# Autodesk Inventor assembly: 6_right_arm_no error
(part 2 of 2)
Size Designation: M3 x 6
Categories: <MemberInstance><Categories><Category DisplayName="Fasteners" InternalName="e4da775c-781d-43d5-af7c-5136215cf5a6" Mnemonic="FSTN"><Category DisplayName="Bolts" InternalName="536e6df0-f778-49ac-b2f2-25c71d2aa0b2" Mnemonic="SCRW"><CategoryParameter DisplayName="Nominal Diameter Designation" InternalName="03caf894-eafd-4c09-a035-916ac084b87b" Mnemonic="nomdiadesig"/><CategoryParameter DisplayName="Nominal Length" InternalName="238ecbaf-3e6c-45dd-aa95-4068c8e0fd02" Mnemonic="nomlen"/><CategoryParameter DisplayName="Thread Designation" InternalName="586d5e89-370a-4089-914f-0110033585c7" Mnemonic="thrdesign"/><CategoryParameter DisplayName="Thread Series Designation" InternalName="87c5849c-b3a5-4c3e-9c9b-2feecef9be86" Mnemonic="thrserdsgn"/><CategoryParameter DisplayName="Nominal Diameter" InternalName="8bbe3f8e-44cf-40a9-a251-3a6edc8168d6" Mnemonic="nomdia"/><CategoryParameter DisplayName="Thread Type" InternalName="b4bbb7bc-d6aa-4c9f-a9a9-4152b9f6fe49" Mnemonic="thrtype"/><CategoryParameter DisplayName="Thread Pitch" InternalName="bb82302e-82d8-4176-8fc1-c5d7bb17d5ad" Mnemonic="pitch1"/><CategoryParameter DisplayName="Threads per Unit" InternalName="bdc6e7d2-ffd0-4d9c-a173-16b95ebb912d" Mnemonic="thrperunit1"/><CategoryParameter DisplayName="Thread Class" InternalName="ebc0d23b-2cc6-4d2a-b376-d52aae53bab6" Mnemonic="thrclss"/><Category DisplayName="Round Head" InternalName="df3578aa-538f-4805-96a8-2439eb0c3cf7" Mnemonic="RNDSCRW"><CategoryParameter DisplayName="Grip Length" InternalName="2c6ace26-543b-4217-91c4-9cdf8c3ec6f1" Mnemonic="grplen"/><CategoryParameter DisplayName="Head Height" InternalName="2d152238-84fe-49ae-94c3-3fee884c292b" Mnemonic="headh"/><CategoryParameter DisplayName="Property Class" InternalName="85496db6-1567-48ed-b0d4-aa1f03366005" Mnemonic="propclss"/><CategoryParameter DisplayName="Thread Length" InternalName="a1e5edc5-4ca7-4847-8786-65b14d35af16" Mnemonic="thrlen"/><CategoryParameter DisplayName="Shank Diameter" InternalName="c22f1a48-b8d5-43ef-ac5e-546ba91c0bd6" Mnemonic="grpdia"/><CategoryParameter DisplayName="Head Diameter" InternalName="e71ee7a1-06fd-425c-ba3b-09769885677c" Mnemonic="headdia"/></Category></Category></Category><Category DisplayName="DataType" InternalName="23b78d0f-2648-40c6-8793-ca6db495c9e8" Mnemonic="DATATYPE"><CategoryParameter DisplayName="DisplayName" InternalName="05415f3d-3907-474b-a020-eb9d644f4cf3" Mnemonic="DISPLAYNAME"/><CategoryParameter DisplayName="Standard" InternalName="0c0a119c-1e12-4c84-803f-101930972f5e" Mnemonic="STANDARD"/><CategoryParameter DisplayName="Description" InternalName="13903e3d-64b1-4950-80da-f627842ea37f" Mnemonic="DESCRIPTION"/><CategoryParameter DisplayName="Designation" InternalName="2675968c-4ce5-49e0-a4f5-552d29089031" Mnemonic="DESIGNATION"/><CategoryParameter DisplayName="Default Row" InternalName="2af9ec52-faaa-4026-b378-f9fa4afca842" Mnemonic="DEFAULTROW"/><CategoryParameter DisplayName="Folder Name" InternalName="3f06958e-8713-4116-9be7-ed6184ecc97b" Mnemonic="FOLDERNAME"/><CategoryParameter DisplayName="Revision Guid" InternalName="45a75005-10b1-4dfc-8d6d-dfe629f0b93c" Mnemonic="REVISIONGUID"/><CategoryParameter DisplayName="FileName" InternalName="8b46a4cc-9585-4fed-90c3-899f57e09a73" Mnemonic="FILENAME"/><CategoryParameter DisplayName="StdsOrg" InternalName="8f5914e1-4693-403f-8ab5-d37768198c9d" Mnemonic="STDSORG"/><CategoryParameter DisplayName="Family Version" InternalName="914462f6-6e19-4b14-ba84-155b9680b1d0" Mnemonic="FAMILYREVISION"/><CategoryParameter DisplayName="Standard Revision" InternalName="91d5a463-65c2-4fde-b823-3b7fea5e8e17" Mnemonic="STANDARDREVISION"/><CategoryParameter DisplayName="Member Revision" InternalName="a65d44b9-392f-4f4f-857b-e4b3d54996fe" Mnemonic="MEMBERREVISION"/><CategoryParameter DisplayName="ClipFormat" InternalName="bc51e27b-3422-4e78-93ef-cec197ddf230" Mnemonic="CLIPFORMAT"/><CategoryParameter DisplayName="Manufacturer" InternalName="cd6c7a72-a28a-4e50-99a9-2c7f4e13e5ad" Mnemonic="MANUFACTURER"/><CategoryParameter DisplayName="InternalName" InternalName="cf1d0246-76d9-4b4a-8305-fa0409afb5c1" Mnemonic="INTERNALNAME"/><CategoryParameter DisplayName="IsMetric" InternalName="e2385c5b-1ea4-4823-96a8-8de651266ec3" Mnemonic="ISMETRIC"/><Category DisplayName="Part" InternalName="c0e0b642-3bcb-4cc8-9e80-f96d35c4afa4" Mnemonic="PART"><CategoryParameter DisplayName="Part Number" InternalName="016b6077-bfbe-49bd-92c9-d8d59c39c941" Mnemonic="PARTNUMBER"/><CategoryParameter DisplayName="Stock Number" InternalName="4dba7c1c-e26c-444e-836c-b08b433409a8" Mnemonic="STOCKNUMBER"/><CategoryParameter DisplayName="Material Key" InternalName="5c9a8adb-dd2b-4535-b97f-0a94a95fe41f" Mnemonic="MATERIALKEY"/><CategoryParameter DisplayName="Material" InternalName="818a152a-d3c3-49ca-80ee-df7d91421b8e" Mnemonic="MATERIAL"/></Category></Category><Category DisplayName="LegacyMap" InternalName="cd87c42b-3e48-431e-b5c0-1cbeb14dfe77" Mnemonic="LEGACYMAP"><CategoryParameter DisplayName="unique DA member ID" InternalName="0918ad47-427f-4fed-ae26-24c81c58f590" Mnemonic="DACOOKIE"/><CategoryParameter DisplayName="Merge11 ID" InternalName="0ee8fb18-e2ed-4f39-96f6-1f4b5f50aa71" Mnemonic="MERGE11"/><CategoryParameter DisplayName="unique CC member ID" InternalName="5193edd4-b2b0-4ab4-9d54-de900eee34e0" Mnemonic="CCCOOKIE"/><CategoryParameter DisplayName="Split ID" InternalName="72b5c83c-be7f-45c4-ae51-9160ea6deb26" Mnemonic="SPLIT"/><CategoryParameter DisplayName="MemberID" InternalName="8e5e0294-fc51-4c8f-b3d7-003dc5ed94f6" Mnemonic="MEMBERID"/><CategoryParameter DisplayName="CatalogName" InternalName="d99d1e27-aa94-4de2-af4c-c348882a6f4f" Mnemonic="CATALOGNAME"/><CategoryParameter DisplayName="FamilyNumber" InternalName="e705e1f4-09cb-413e-91f9-551b4188271e" Mnemonic="FAMILYNUMBER"/></Category></Categories><FamilyTemplate Id="si0145"><FamilyTemplateParameters><FamilyTemplateParameter ObjectType="kUserParameterObject" ValueType="xs:double" Id="1" ObjectReferenceKey="GUL"/><FamilyTemplateParameter ObjectType="kUserParameterObject" ValueType="xs:double" Id="2" ObjectReferenceKey="SPD"/><FamilyTemplateParameter ObjectType="kUserParameterObject" ValueType="xs:double" Id="3" ObjectReferenceKey="NLG"/><FamilyTemplateParameter ObjectType="kUserParameterObject" ValueType="xs:double" Id="4" ObjectReferenceKey="TPU"/><FamilyTemplateParameter ObjectType="kUserParameterObject" ValueType="xs:double" Id="5" ObjectReferenceKey="TOA"/><FamilyTemplateParameter ObjectType="kUserParameterObject" ValueType="xs:double" Id="6" ObjectReferenceKey="GD1"/><FamilyTemplateParameter ObjectType="kUserParameterObject" ValueType="xs:double" Id="7" ObjectReferenceKey="GEL"/><FamilyTemplateParameter ObjectType="kUserParameterObject" ValueType="xs:double" Id="8" ObjectReferenceKey="SW"/><FamilyTemplateParameter ObjectType="kUserParameterObject" ValueType="xs:double" Id="9" ObjectReferenceKey="THREADDIA"/><FamilyTemplateParameter ObjectType="kUserParameterObject" ValueType="xs:double" Id="10" ObjectReferenceKey="INTI"/><FamilyTemplateParameter ObjectType="kUserParameterObject" ValueType="xs:double" Id="11" ObjectReferenceKey="BDM"/><FamilyTemplateParameter ObjectType="kUserParameterObject" ValueType="xs:double" Id="12" ObjectReferenceKey="RR"/><FamilyTemplateParameter ObjectType="kUserParameterObject" ValueType="xs:double" Id="13" ObjectReferenceKey="KOH"/><FamilyTemplateParameter ObjectType="kUserParameterObject" ValueType="xs:double" Id="14" ObjectReferenceKey="PTC"/><FamilyTemplateParameter ObjectType="kUserParameterObject" ValueType="xs:double" Id="15" ObjectReferenceKey="KOD"/><FamilyTemplateParameter ObjectType="kUserParameterObject" ValueType="xs:double" Id="16" ObjectReferenceKey="NND"/><FamilyTemplateParameter ObjectType="kUserParameterObject" ValueType="xs:double" Id="17" ObjectReferenceKey="GD"/><FamilyTemplateParameter ObjectType="kUserParameterObject" ValueType="xs:double" Id="18" ObjectReferenceKey="GAL"/><FamilyTemplateParameter ObjectType="kUserParameterObject" ValueType="xs:double" Id="19" ObjectReferenceKey="KOH1"/><FamilyTemplateParameter ObjectType="kUserParameterObject" ValueType="xs:double" Id="20" ObjectReferenceKey="E0"/><FamilyTemplateParameter ObjectType="kUserParameterObject" ValueType="xs:double" Id="132" ObjectReferenceKey="R"/><FamilyTemplateParameter ObjectType="kPropertyObject" ValueType="xs:string" Id="100" ObjectReferenceKey="{32853F0F-3444-11d1-9E93-0060B03C1CA6}" SubObjectId="52"/><FamilyTemplateParameter ObjectType="kPropertyObject" ValueType="xs:string" Id="105" ObjectReferenceKey="{32853F0F-3444-11d1-9E93-0060B03C1CA6}" SubObjectId="5"/><FamilyTemplateParameter ObjectType="kPartComponentDefinitionObject" ValueType="xs:string" Id="110" SubObjectId="Material"/><FamilyTemplateParameter ObjectType="kThreadFeatureObject" ValueType="xs:structure" Id="300" ObjectReferenceKey="1002000010000000a2070000000000008000000000000000" SubObjectId="ThreadInfo"><FamilyTemplateParameter ObjectType="" ValueType="xs:string" Id="301" SubObjectId="ThreadDesignation"/><FamilyTemplateParameter ObjectType="" ValueType="xs:string" Id="302" SubObjectId="ThreadType"/><FamilyTemplateParameter ObjectType="" ValueType="xs:string" Id="303" SubObjectId="ThreadClass"/></FamilyTemplateParameter></FamilyTemplateParameters></FamilyTemplate><CategoryParameterMap><ParamToTemplateMap><ParamToTemplate CategoryParameter="//CategoryParameter[@InternalName='05415f3d-3907-474b-a020-eb9d644f4cf3']" ConstantValue="ISO 7380-1"/><ParamToTemplate CategoryParameter="//CategoryParameter[@InternalName='cf1d0246-76d9-4b4a-8305-fa0409afb5c1']" ConstantValue="7e948a18-7d98-46c8-9f69-82be43869b08"/><ParamToTemplate CategoryParameter="//CategoryParameter[@InternalName='3f06958e-8713-4116-9be7-ed6184ecc97b']" ConstantValue="ISO 7380-1"/><ParamToTemplate CategoryParameter="//CategoryParameter[@InternalName='914462f6-6e19-4b14-ba84-155b9680b1d0']" ConstantValue="10"/><ParamToTemplate CategoryParameter="//CategoryParameter[@InternalName='bc51e27b-3422-4e78-93ef-cec197ddf230']" ConstantValue="CF_INVENTOR.STDPARTS"/><ParamToTemplate CategoryParameter="//CategoryParameter[@InternalName='e2385c5b-1ea4-4823-96a8-8de651266ec3']" ConstantValue="true"/><ParamToTemplate CategoryParameter="//CategoryParameter[@InternalName='13903e3d-64b1-4950-80da-f627842ea37f']" ConstantValue="Hexagon Socket Button Head Screw - Product grade A"/><ParamToTemplate CategoryParameter="//CategoryParameter[@InternalName='8f5914e1-4693-403f-8ab5-d37768198c9d']" ConstantValue="ISO"/><ParamToTemplate CategoryParameter="//CategoryParameter[@InternalName='0c0a119c-1e12-4c84-803f-101930972f5e']" ConstantValue="ISO 7380-1"/><ParamToTemplate CategoryParameter="//CategoryParameter[@InternalName='cd6c7a72-a28a-4e50-99a9-2c7f4e13e5ad']" TemplateParameter="104"/><ParamToTemplate CategoryParameter="//CategoryParameter[@InternalName='91d5a463-65c2-4fde-b823-3b7fea5e8e17']" ConstantValue="First edition 2011-08-01"/><ParamToTemplate CategoryParameter="//CategoryParameter[@InternalName='45a75005-10b1-4dfc-8d6d-dfe629f0b93c']" ConstantValue="28e2f25c-6dc8-4906-99e1-9c4ceb92a97a"/><ParamToTemplate CategoryParameter="//CategoryParameter[@InternalName='2af9ec52-faaa-4026-b378-f9fa4afca842']" ConstantValue="10"/><ParamToTemplate CategoryParameter="//CategoryParameter[@InternalName='d99d1e27-aa94-4de2-af4c-c348882a6f4f']" ConstantValue="ISO"/><ParamToTemplate CategoryParameter="//CategoryParameter[@InternalName='e705e1f4-09cb-413e-91f9-551b4188271e']" ConstantValue="16"/><ParamToTemplate CategoryParameter="//CategoryParameter[@InternalName='8b46a4cc-9585-4fed-90c3-899f57e09a73']" ConstantValue="ISO 7380-1 - M3 x 6"/><ParamToTemplate CategoryParameter="//CategoryParameter[@InternalName='a65d44b9-392f-4f4f-857b-e4b3d54996fe']" ConstantValue="06E58314-F7E5-4B9F-9F34-16689E4488C2"/><ParamToTemplate CategoryParameter="//CategoryParameter[@InternalName='2c6ace26-543b-4217-91c4-9cdf8c3ec6f1']" ConstantValue="1.5"/><ParamToTemplate CategoryParameter="//CategoryParameter[@InternalName='ebc0d23b-2cc6-4d2a-b376-d52aae53bab6']" ConstantValue="6g"/><ParamToTemplate CategoryParameter="//CategoryParameter[@InternalName='03caf894-eafd-4c09-a035-916ac084b87b']" ConstantValue="M3"/><ParamToTemplate CategoryParameter="//CategoryParameter[@InternalName='b4bbb7bc-d6aa-4c9f-a9a9-4152b9f6fe49']" ConstantValue="ISO Metric profile"/><ParamToTemplate CategoryParameter="//CategoryParameter[@InternalName='8e5e0294-fc51-4c8f-b3d7-003dc5ed94f6']" ConstantValue="10"/><ParamToTemplate CategoryParameter="//CategoryParameter[@InternalName='c22f1a48-b8d5-43ef-ac5e-546ba91c0bd6']" TemplateParameter="11"/><ParamToTemplate CategoryParameter="//CategoryParameter[@InternalName='2675968c-4ce5-49e0-a4f5-552d29089031']" TemplateParameter="100"/><ParamToTemplate CategoryParameter="//CategoryParameter[@InternalName='a1e5edc5-4ca7-4847-8786-65b14d35af16']" TemplateParameter="7"/><ParamToTemplate CategoryParameter="//CategoryParameter[@InternalName='e71ee7a1-06fd-425c-ba3b-09769885677c']" TemplateParameter="15"/><ParamToTemplate CategoryParameter="//CategoryParameter[@InternalName='2d152238-84fe-49ae-94c3-3fee884c292b']" TemplateParameter="13"/><ParamToTemplate CategoryParameter="//CategoryParameter[@InternalName='818a152a-d3c3-49ca-80ee-df7d91421b8e']" TemplateParameter="110"/><ParamToTemplate CategoryParameter="//CategoryParameter[@InternalName='238ecbaf-3e6c-45dd-aa95-4068c8e0fd02']" TemplateParameter="3"/><ParamToTemplate CategoryParameter="//CategoryParameter[@InternalName='8bbe3f8e-44cf-40a9-a251-3a6edc8168d6']" TemplateParameter="16"/><ParamToTemplate CategoryParameter="//CategoryParameter[@InternalName='016b6077-bfbe-49bd-92c9-d8d59c39c941']" TemplateParameter="105"/><ParamToTemplate CategoryParameter="//CategoryParameter[@InternalName='bb82302e-82d8-4176-8fc1-c5d7bb17d5ad']" TemplateParameter="14"/><ParamToTemplate CategoryParameter="//CategoryParameter[@InternalName='586d5e89-370a-4089-914f-0110033585c7']" TemplateParameter="301"/><ParamToTemplate CategoryParameter="//CategoryParameter[@InternalName='bdc6e7d2-ffd0-4d9c-a173-16b95ebb912d']" TemplateParameter="4"/></ParamToTemplateMap></CategoryParameterMap></MemberInstance>
Density: 8 g/cm^3
Appearance: Default
Sending System: Autodesk Inventor 2026
Author: chanh
## Documents named in this file (28)
- C:\Users\LG\Desktop\RHp_Humanoid_ver1\Assembly\6_right_arm.iam
- C:\Users\LG\Desktop\RHp_Humanoid_ver1\Part\HTD-45H, Horn\HTD-45H\HTD-45H.iam
- C:\Users\LG\Desktop\RHp_Humanoid_ver1\Part\HTD-45H, Horn\Horn\Top Horn.ipt
- C:\Users\LG\Desktop\RHp_Humanoid_ver1\Part\Frame\Arm\axis_18_top_frame.ipt
- C:\Users\LG\Desktop\RHp_Humanoid_ver1\Part\HTD-45H, Horn\Horn\Bottom Horn.ipt
- C:\Users\LG\Desktop\RHp_Humanoid_ver1\Part\Frame\Arm\axis_19_bottom_frame.ipt
- C:\Users\LG\Desktop\RHp_Humanoid_ver1\Part\Frame\Arm\axis_20_top_frame.ipt
- C:\Users\LG\Desktop\RHp_Humanoid_ver1\Part\Bolt, Bearing, Nut, Washer\2030 Teflon Sheet.ipt
- C:\Users\LG\Desktop\RHp_Humanoid_ver1\Part\Frame\Arm\axis_20_bottom_frame.ipt
- C:\Users\LG\Desktop\RHp_Humanoid_ver1\Part\Frame\Arm\axis_21_top_frame.ipt
- C:\Users\LG\Desktop\RHp_Humanoid_ver1\Part\Frame\Arm\axis_21_bottom_frame.ipt
- C:\Users\LG\Desktop\RHp_Humanoid_ver1\Part\Frame\Arm\axis_22_bottom_frame.ipt
- C:\Users\LG\Desktop\RHp_Humanoid_ver1\Part\Frame\Arm\axis_22_top_frame.ipt
- C:\Users\LG\Desktop\RHp_Humanoid_ver1\Part\Frame\Arm\HTD-45H_no bottom horn.ipt
- C:\Users\LG\Desktop\RHp_Humanoid_ver1\Part\Frame\Arm\gripper_frame.ipt
- **C:\Users\LG\Desktop\RHp_Humanoid_ver1\Assembly\6_right_arm.iam*LocalDocs*xAaaaqlbaAaaaaaaaAaaaqn4s4f*M2x4 Bolt.ipt
- **C:\Users\LG\Desktop\RHp_Humanoid_ver1\Assembly\6_right_arm.iam*LocalDocs*xAaaaaedaAaaaaaaaAaaaaugyFa*M3x6 Bolt.ipt
- C:\Users\LG\Desktop\RHp_Humanoid_ver1\Part\Bolt, Bearing, Nut, Washer\볼트, 너트\M3 Nut.ipt
- **C:\Users\LG\Desktop\RHp_Humanoid_ver1\Assembly\6_right_arm.iam*LocalDocs*xAaaaa5baAaaaaaaaAaaaqdxtGe*M2x6 Bolt.ipt
- **C:\Users\LG\Desktop\RHp_Humanoid_ver1\Assembly\6_right_arm.iam*LocalDocs*xAaaaqfdaAaaaaaaaAaaaqi4sPf*M3x8 Bolt.ipt
- C:\Users\LG\Desktop\RHp_Humanoid_ver1\Part\Bolt, Bearing, Nut, Washer\볼트, 너트\M2x4 Bolt.ipt
- C:\Users\LG\Desktop\RHp_Humanoid_ver1\Part\Bolt, Bearing, Nut, Washer\볼트, 너트\M3x6 Bolt.ipt
- C:\Users\LG\Desktop\RHp_Humanoid_ver1\Part\Bolt, Bearing, Nut, Washer\볼트, 너트\M2x6 Bolt.ipt
- C:\Users\LG\Desktop\RHp_Humanoid_ver1\Part\Bolt, Bearing, Nut, Washer\볼트, 너트\M3x8 Bolt.ipt
- **C:\Users\LG\Desktop\RHp_Humanoid_ver1\Assembly\6_right_arm_no error.iam*LocalDocs*xAaaaaedaAaaaaaaaAaaaaugyFa*M3x6 Bolt.ipt
- **C:\Users\LG\Desktop\RHp_Humanoid_ver1\Assembly\6_right_arm_no error.iam*LocalDocs*xAaaaa5baAaaaaaaaAaaaqdxtGe*M2x6 Bolt.ipt
- **C:\Users\LG\Desktop\RHp_Humanoid_ver1\Assembly\6_right_arm_no error.iam*LocalDocs*xAaaaqfdaAaaaaaaaAaaaqi4sPf*M3x8 Bolt.ipt
- **C:\Users\LG\Desktop\RHp_Humanoid_ver1\Assembly\6_right_arm_no error.iam*LocalDocs*xAaaaqlbaAaaaaaaaAaaaqn4s4f*M2x4 Bolt.ipt
## Components (107 placed, 18 different names)
1. M2x4 Bolt:21 — Rigid:22
2. M2x4 Bolt:20 — Rigid:21
3. M2x4 Bolt:19 — Rigid:20
4. M2x4 Bolt:18 — Rigid:19
5. M2x4 Bolt:6 — Rigid:6
6. M2x4 Bolt:8 — Rigid:2
7. M2x4 Bolt:7 — Rigid:3
8. M2x4 Bolt:9 — Rigid:4
9. M2x4 Bolt:1 — Rigid:5
10. M2x4 Bolt:10 — Rigid:12
11. M2x4 Bolt:11 — Rigid:13
12. M2x4 Bolt:17 — Rigid:11
13. M2x4 Bolt:16 — Rigid:14
14. axis_18_top_frame:1 — Mate:6, Mate:7, Mate:8, Mate:9, Mate:14, Mate:15, Rigid:2, Rigid:3, Rigid:4, Rigid:5, Rigid:6, Rigid:11, Rigid:12, Rigid:13, Rigid:14, Rigid:19, Rigid:20, Rigid:21, Rigid:22
15. Top Horn:1 — Mate:6, Mate:14, Mate:15
16. M2x4 Bolt:2 — Rigid:7
17. M2x4 Bolt:4 — Rigid:9
18. M2x4 Bolt:5 — Rigid:8
19. M2x4 Bolt:3 — Rigid:10
20. M2x4 Bolt:13 — Rigid:15
21. M2x4 Bolt:12 — Rigid:17
22. M2x4 Bolt:15 — Rigid:18
23. M2x4 Bolt:14 — Rigid:16
24. M2x4 Bolt:55 — Rigid:96
25. M2x4 Bolt:56 — Rigid:98
26. M2x4 Bolt:57 — Rigid:95
27. M2x4 Bolt:58 — Rigid:97
28. axis_19_bottom_frame:1 — Flush:2, Mate:12, Mate:13, Rigid:7, Rigid:8, Rigid:9, Rigid:10, Rigid:15, Rigid:16, Rigid:17, Rigid:18, Mate:49, Mate:50, Flush:15, Rigid:95, Rigid:96, Rigid:97, Rigid:98
29. Bottom Horn:1 — Mate:10, Mate:11, Flush:1
30. Top Horn:2 — Rotational:2, Flush:2, Mate:12, Mate:13
31. HTD-45H:2 [sub-assembly] — Mate:7, Mate:8, Mate:9, Rotational:2, Mate:10, Mate:11, Flush:1
32. 2030 Teflon Sheet:1 — Mate:19, Mate:20, Mate:21, Mate:24, Mate:25
33. 2030 Teflon Sheet:2 — Mate:24, Mate:25, Mate:26
34. M2x4 Bolt:27 — Rigid:27
35. M2x4 Bolt:28 — Rigid:29
36. M2x4 Bolt:29 — Rigid:30
37. M2x4 Bolt:26 — Rigid:28
38. axis_20_top_frame:1 — Mate:19, Mate:20, Mate:21, Mate:47, Flush:14, Mate:48
39. axis_20_bottom_frame:1 — Mate:22, Flush:6, Mate:23, Mate:26, Mate:29, Mate:30, Mate:31, Rigid:27, Rigid:28, Rigid:29, Rigid:30, Rigid:31, Rigid:32, Rigid:33, Rigid:34, Rigid:35, Rigid:36, Rigid:37, Rigid:38
40. Top Horn:3 — Mate:22, Flush:6, Mate:23, Rotational:6
41. HTD-45H:6 — Rotational:6, Mate:47, Flush:14, Mate:48, Mate:49, Mate:50, Flush:15
42. M2x4 Bolt:30 — Rigid:31
43. M2x4 Bolt:31 — Rigid:32
44. M2x4 Bolt:33 — Rigid:33
45. M2x4 Bolt:32 — Rigid:34
46. M2x4 Bolt:34 — Rigid:35
47. M2x4 Bolt:35 — Rigid:37
48. M2x4 Bolt:36 — Rigid:36
49. M2x4 Bolt:37 — Rigid:38
50. M2x4 Bolt:43 — Rigid:44
51. M2x4 Bolt:44 — Rigid:45
52. M2x4 Bolt:45 — Rigid:46
53. M2x4 Bolt:46 — Rigid:47
54. M2x4 Bolt:39 — Rigid:40
55. M2x4 Bolt:38 — Rigid:39
56. M2x4 Bolt:41 — Rigid:42
57. M2x4 Bolt:40 — Rigid:41
58. M2x4 Bolt:42 — Rigid:43
59. M3 Nut:3 — Rigid:64
60. M3 Nut:4 — Rigid:62
61. M3 Nut:2 — Rigid:63
62. M3 Nut:1 — Rigid:61
63. M3x6 Bolt:1 — Rigid:58
64. M3x6 Bolt:2 — Rigid:59
65. M3x6 Bolt:3 — Rigid:60
66. M3x6 Bolt:4 — Rigid:57
67. axis_21_top_frame:1 — Mate:36, Mate:37, Mate:38, Mate:39, Mate:45, Rigid:39, Rigid:40, Rigid:41, Rigid:42, Rigid:43, Rigid:44, Rigid:45, Rigid:46, Rigid:47, Rigid:57, Rigid:58, Rigid:59, Rigid:60
68. axis_21_bottom_frame:1 — Mate:39, Mate:40, Flush:10, Mate:44, Flush:11, Rigid:61, Rigid:62, Rigid:63, Rigid:64
69. Bottom Horn:2 — Mate:27, Flush:7, Mate:28
70. Top Horn:4 — Rotational:4, Mate:29, Mate:30, Mate:31
71. HTD-45H:4 [sub-assembly] — Mate:27, Flush:7, Mate:28, Rotational:4, Mate:35, Flush:8, Flush:9, Mate:37, Mate:38
72. M2x4 Bolt:47 — Rigid:65
73. M2x4 Bolt:49 — Rigid:66
74. M2x4 Bolt:50 — Rigid:68
75. M2x4 Bolt:48 — Rigid:67
76. M2x4 Bolt:54 — Rigid:69
77. M2x4 Bolt:51 — Rigid:70
78. M2x4 Bolt:53 — Rigid:72
79. M2x4 Bolt:52 — Rigid:71
80. M2x6 Bolt:5 — Rigid:77
81. M2x6 Bolt:7 — Rigid:78
82. M2x6 Bolt:6 — Rigid:79
83. M2x6 Bolt:8 — Rigid:80
84. M2x6 Bolt:9 — Rigid:81
85. M2x6 Bolt:2 — Rigid:74
86. M2x6 Bolt:1 — Rigid:73
87. M2x6 Bolt:3 — Rigid:76
88. M2x6 Bolt:4 — Rigid:75
89. M3x8 Bolt:4 — Rigid:88
90. M3x8 Bolt:5 — Rigid:89
91. M3x8 Bolt:6 — Rigid:90
92. M3 Nut:10 — Rigid:93
93. M3 Nut:9 — Rigid:92
94. M3 Nut:8 — Rigid:91
95. M3x8 Bolt:3 — Rigid:84
96. M3x8 Bolt:2 — Rigid:83
97. M3x8 Bolt:1 — Rigid:82
98. M3 Nut:6 — Rigid:87
99. M3 Nut:7 — Rigid:86
100. M3 Nut:5 — Rigid:85
101. axis_22_bottom_frame:1 — Mate:41, Mate:42, Mate:43, Rigid:1, Rigid:65, Rigid:66, Rigid:67, Rigid:68, Rigid:69, Rigid:70, Rigid:71, Rigid:72, Rigid:85, Rigid:86, Rigid:87
102. axis_22_top_frame:1 — Mate:44, Flush:11, Mate:45, Rigid:73, Rigid:74, Rigid:75, Rigid:76, Rigid:77, Rigid:78, Rigid:79, Rigid:80, Rigid:81, Rigid:91, Rigid:92, Rigid:93, Rigid:94
103. gripper_frame:1 — Rigid:1, Rigid:82, Rigid:83, Rigid:84
104. gripper_frame:2 — Rigid:88, Rigid:89, Rigid:90, Rigid:94
105. Top Horn:5 — Rotational:5, Mate:41, Mate:42, Mate:43
106. Bottom Horn:3 — Mate:32, Mate:33, Mate:34
107. HTD-45H:5 [sub-assembly] — Rotational:5, Mate:32, Mate:33, Mate:34, Mate:35, Flush:8, Flush:9, Mate:36, Mate:40, Flush:10
## Relationships (140: WeldJoint 85, Mate 41, Flush 10, RevoluteJoint 4)
- Rotational:2 [RevoluteJoint]: Top Horn:2 ↔ HTD-45H:2
- Rotational:4 [RevoluteJoint]: Top Horn:4 ↔ HTD-45H:4
- Rotational:5 [RevoluteJoint]: Top Horn:5 ↔ HTD-45H:5
- Rotational:6 [RevoluteJoint]: Top Horn:3 ↔ HTD-45H:6
- Mate:6: axis_18_top_frame:1 ↔ Top Horn:1
- Mate:7: axis_18_top_frame:1 ↔ HTD-45H:2
- Mate:8 (2.5 mm): axis_18_top_frame:1 ↔ HTD-45H:2
- Mate:9: axis_18_top_frame:1 ↔ HTD-45H:2
- Mate:10: Bottom Horn:1 ↔ HTD-45H:2
- Mate:11: Bottom Horn:1 ↔ HTD-45H:2
- Flush:1: Bottom Horn:1 ↔ HTD-45H:2
- Flush:2 (14.5 mm): axis_19_bottom_frame:1 ↔ Top Horn:2
- Mate:12: axis_19_bottom_frame:1 ↔ Top Horn:2
- Mate:13: axis_19_bottom_frame:1 ↔ Top Horn:2
- Mate:14: axis_18_top_frame:1 ↔ Top Horn:1
- Mate:15: axis_18_top_frame:1 ↔ Top Horn:1
- Mate:19: 2030 Teflon Sheet:1 ↔ axis_20_top_frame:1
- Mate:20: 2030 Teflon Sheet:1 ↔ axis_20_top_frame:1
- Mate:21: 2030 Teflon Sheet:1 ↔ axis_20_top_frame:1
- Mate:22: axis_20_bottom_frame:1 ↔ Top Horn:3
- Flush:6: axis_20_bottom_frame:1 ↔ Top Horn:3
- Mate:23: axis_20_bottom_frame:1 ↔ Top Horn:3
- Mate:24: 2030 Teflon Sheet:1 ↔ 2030 Teflon Sheet:2
- Mate:25: 2030 Teflon Sheet:1 ↔ 2030 Teflon Sheet:2
- Mate:26: 2030 Teflon Sheet:2 ↔ axis_20_bottom_frame:1
- Mate:27: Bottom Horn:2 ↔ HTD-45H:4
- Flush:7: Bottom Horn:2 ↔ HTD-45H:4
- Mate:28: Bottom Horn:2 ↔ HTD-45H:4
- Mate:29 (30.43 mm): axis_20_bottom_frame:1 ↔ Top Horn:4
- Mate:30 (-14 mm): axis_20_bottom_frame:1 ↔ Top Horn:4
- Mate:31: axis_20_bottom_frame:1 ↔ Top Horn:4
- Mate:32: Bottom Horn:3 ↔ HTD-45H:5
- Mate:33: Bottom Horn:3 ↔ HTD-45H:5
- Mate:34: Bottom Horn:3 ↔ HTD-45H:5
- Mate:35: HTD-45H:4 ↔ HTD-45H:5
- Flush:8: HTD-45H:4 ↔ HTD-45H:5
- Flush:9: HTD-45H:4 ↔ HTD-45H:5
- Mate:36 (5 mm): axis_21_top_frame:1 ↔ HTD-45H:5
- Mate:37: axis_21_top_frame:1 ↔ HTD-45H:4
- Mate:38: axis_21_top_frame:1 ↔ HTD-45H:4
- Mate:39: axis_21_top_frame:1 ↔ axis_21_bottom_frame:1
- Mate:40: axis_21_bottom_frame:1 ↔ HTD-45H:5
- Flush:10: axis_21_bottom_frame:1 ↔ HTD-45H:5
- Mate:41: axis_22_bottom_frame:1 ↔ Top Horn:5
- Mate:42: axis_22_bottom_frame:1 ↔ Top Horn:5
- Mate:43 (19.43 mm): axis_22_bottom_frame:1 ↔ Top Horn:5
- Mate:44: axis_21_bottom_frame:1 ↔ axis_22_top_frame:1
- Flush:11: axis_21_bottom_frame:1 ↔ axis_22_top_frame:1
- Mate:45: axis_21_top_frame:1 ↔ axis_22_top_frame:1
- Mate:47: axis_20_top_frame:1 ↔ HTD-45H:6
- Flush:14: axis_20_top_frame:1 ↔ HTD-45H:6
- Mate:48: axis_20_top_frame:1 ↔ HTD-45H:6
- Rigid:1 [WeldJoint]: axis_22_bottom_frame:1 ↔ gripper_frame:1
- Rigid:2 [WeldJoint]: M2x4 Bolt:8 ↔ axis_18_top_frame:1
- Rigid:3 [WeldJoint]: M2x4 Bolt:7 ↔ axis_18_top_frame:1
- Rigid:4 [WeldJoint]: M2x4 Bolt:9 ↔ axis_18_top_frame:1
- Rigid:5 [WeldJoint]: M2x4 Bolt:1 ↔ axis_18_top_frame:1
- Rigid:6 [WeldJoint]: M2x4 Bolt:6 ↔ axis_18_top_frame:1
- Rigid:7 [WeldJoint]: M2x4 Bolt:2 ↔ axis_19_bottom_frame:1
- Rigid:8 [WeldJoint]: M2x4 Bolt:5 ↔ axis_19_bottom_frame:1
- Rigid:9 [WeldJoint]: M2x4 Bolt:4 ↔ axis_19_bottom_frame:1
- Rigid:10 [WeldJoint]: M2x4 Bolt:3 ↔ axis_19_bottom_frame:1
- Rigid:11 [WeldJoint]: M2x4 Bolt:17 ↔ axis_18_top_frame:1
- Rigid:12 [WeldJoint]: M2x4 Bolt:10 ↔ axis_18_top_frame:1
- Rigid:13 [WeldJoint]: M2x4 Bolt:11 ↔ axis_18_top_frame:1
- Rigid:14 [WeldJoint]: M2x4 Bolt:16 ↔ axis_18_top_frame:1
- Rigid:15 [WeldJoint]: M2x4 Bolt:13 ↔ axis_19_bottom_frame:1
- Rigid:16 [WeldJoint]: M2x4 Bolt:14 ↔ axis_19_bottom_frame:1
- Rigid:17 [WeldJoint]: M2x4 Bolt:12 ↔ axis_19_bottom_frame:1
- Rigid:18 [WeldJoint]: M2x4 Bolt:15 ↔ axis_19_bottom_frame:1
- Rigid:19 [WeldJoint]: M2x4 Bolt:18 ↔ axis_18_top_frame:1
- Rigid:20 [WeldJoint]: M2x4 Bolt:19 ↔ axis_18_top_frame:1
- Rigid:21 [WeldJoint]: M2x4 Bolt:20 ↔ axis_18_top_frame:1
- Rigid:22 [WeldJoint]: M2x4 Bolt:21 ↔ axis_18_top_frame:1
- Rigid:27 [WeldJoint]: M2x4 Bolt:27 ↔ axis_20_bottom_frame:1
- Rigid:28 [WeldJoint]: M2x4 Bolt:26 ↔ axis_20_bottom_frame:1
- Rigid:29 [WeldJoint]: M2x4 Bolt:28 ↔ axis_20_bottom_frame:1
- Rigid:30 [WeldJoint]: M2x4 Bolt:29 ↔ axis_20_bottom_frame:1
- Rigid:31 [WeldJoint]: axis_20_bottom_frame:1 ↔ M2x4 Bolt:30
- Rigid:32 [WeldJoint]: axis_20_bottom_frame:1 ↔ M2x4 Bolt:31
- Rigid:33 [WeldJoint]: axis_20_bottom_frame:1 ↔ M2x4 Bolt:33
- Rigid:34 [WeldJoint]: axis_20_bottom_frame:1 ↔ M2x4 Bolt:32
- Rigid:35 [WeldJoint]: axis_20_bottom_frame:1 ↔ M2x4 Bolt:34
- Rigid:36 [WeldJoint]: axis_20_bottom_frame:1 ↔ M2x4 Bolt:36
- Rigid:37 [WeldJoint]: axis_20_bottom_frame:1 ↔ M2x4 Bolt:35
- Rigid:38 [WeldJoint]: axis_20_bottom_frame:1 ↔ M2x4 Bolt:37
- Rigid:39 [WeldJoint]: M2x4 Bolt:38 ↔ axis_21_top_frame:1
- Rigid:40 [WeldJoint]: M2x4 Bolt:39 ↔ axis_21_top_frame:1
- Rigid:41 [WeldJoint]: M2x4 Bolt:40 ↔ axis_21_top_frame:1
- Rigid:42 [WeldJoint]: M2x4 Bolt:41 ↔ axis_21_top_frame:1
- Rigid:43 [WeldJoint]: M2x4 Bolt:42 ↔ axis_21_top_frame:1
- Rigid:44 [WeldJoint]: M2x4 Bolt:43 ↔ axis_21_top_frame:1
- Rigid:45 [WeldJoint]: M2x4 Bolt:44 ↔ axis_21_top_frame:1
- Rigid:46 [WeldJoint]: M2x4 Bolt:45 ↔ axis_21_top_frame:1
- Rigid:47 [WeldJoint]: M2x4 Bolt:46 ↔ axis_21_top_frame:1
- Rigid:57 [WeldJoint]: M3x6 Bolt:4 ↔ axis_21_top_frame:1
- Rigid:58 [WeldJoint]: M3x6 Bolt:1 ↔ axis_21_top_frame:1
- Rigid:59 [WeldJoint]: M3x6 Bolt:2 ↔ axis_21_top_frame:1
- Rigid:60 [WeldJoint]: M3x6 Bolt:3 ↔ axis_21_top_frame:1
- Rigid:61 [WeldJoint]: M3 Nut:1 ↔ axis_21_bottom_frame:1
- Rigid:62 [WeldJoint]: M3 Nut:4 ↔ axis_21_bottom_frame:1
- Rigid:63 [WeldJoint]: M3 Nut:2 ↔ axis_21_bottom_frame:1
- Rigid:64 [WeldJoint]: M3 Nut:3 ↔ axis_21_bottom_frame:1
- Rigid:65 [WeldJoint]: M2x4 Bolt:47 ↔ axis_22_bottom_frame:1
- Rigid:66 [WeldJoint]: M2x4 Bolt:49 ↔ axis_22_bottom_frame:1
- Rigid:67 [WeldJoint]: M2x4 Bolt:48 ↔ axis_22_bottom_frame:1
- Rigid:68 [WeldJoint]: M2x4 Bolt:50 ↔ axis_22_bottom_frame:1
- Rigid:69 [WeldJoint]: M2x4 Bolt:54 ↔ axis_22_bottom_frame:1
- Rigid:70 [WeldJoint]: M2x4 Bolt:51 ↔ axis_22_bottom_frame:1
- Rigid:71 [WeldJoint]: M2x4 Bolt:52 ↔ axis_22_bottom_frame:1
- Rigid:72 [WeldJoint]: M2x4 Bolt:53 ↔ axis_22_bottom_frame:1
- Rigid:73 [WeldJoint]: M2x6 Bolt:1 ↔ axis_22_top_frame:1
- Rigid:74 [WeldJoint]: M2x6 Bolt:2 ↔ axis_22_top_frame:1
- Rigid:75 [WeldJoint]: M2x6 Bolt:4 ↔ axis_22_top_frame:1
- Rigid:76 [WeldJoint]: M2x6 Bolt:3 ↔ axis_22_top_frame:1
- Rigid:77 [WeldJoint]: M2x6 Bolt:5 ↔ axis_22_top_frame:1
- Rigid:78 [WeldJoint]: M2x6 Bolt:7 ↔ axis_22_top_frame:1
- Rigid:79 [WeldJoint]: M2x6 Bolt:6 ↔ axis_22_top_frame:1
- Rigid:80 [WeldJoint]: M2x6 Bolt:8 ↔ axis_22_top_frame:1
- Rigid:81 [WeldJoint]: M2x6 Bolt:9 ↔ axis_22_top_frame:1
- Rigid:82 [WeldJoint]: M3x8 Bolt:1 ↔ gripper_frame:1
- Rigid:83 [WeldJoint]: M3x8 Bolt:2 ↔ gripper_frame:1
- Rigid:84 [WeldJoint]: M3x8 Bolt:3 ↔ gripper_frame:1
- Rigid:85 [WeldJoint]: M3 Nut:5 ↔ axis_22_bottom_frame:1
- Rigid:86 [WeldJoint]: M3 Nut:7 ↔ axis_22_bottom_frame:1
- Rigid:87 [WeldJoint]: M3 Nut:6 ↔ axis_22_bottom_frame:1
- Rigid:88 [WeldJoint]: M3x8 Bolt:4 ↔ gripper_frame:2
- Rigid:89 [WeldJoint]: M3x8 Bolt:5 ↔ gripper_frame:2
- Rigid:90 [WeldJoint]: M3x8 Bolt:6 ↔ gripper_frame:2
- Rigid:91 [WeldJoint]: M3 Nut:8 ↔ axis_22_top_frame:1
- Rigid:92 [WeldJoint]: M3 Nut:9 ↔ axis_22_top_frame:1
- Rigid:93 [WeldJoint]: M3 Nut:10 ↔ axis_22_top_frame:1
- Rigid:94 [WeldJoint]: axis_22_top_frame:1 ↔ gripper_frame:2
- Mate:49: axis_19_bottom_frame:1 ↔ HTD-45H:6
- Mate:50: axis_19_bottom_frame:1 ↔ HTD-45H:6
- Flush:15: axis_19_bottom_frame:1 ↔ HTD-45H:6
- Rigid:95 [WeldJoint]: M2x4 Bolt:57 ↔ axis_19_bottom_frame:1
- Rigid:96 [WeldJoint]: M2x4 Bolt:55 ↔ axis_19_bottom_frame:1
- Rigid:97 [WeldJoint]: M2x4 Bolt:58 ↔ axis_19_bottom_frame:1
- Rigid:98 [WeldJoint]: M2x4 Bolt:56 ↔ axis_19_bottom_frame:1
